# Autodesk Inventor assembly: POM_T5_10
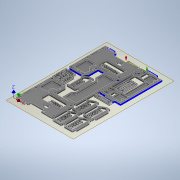
[picture p0: Inventor's stored thumbnail of the model, 180x180]
Saved by Autodesk Inventor 2022 (Build 260153000, 153)
## iProperties
Created: 2022-09-28
Part Number: POM_T5_10
Document SubType Name: Assembly
Designer: Masato
Author: Masato
## Documents named in this file (13)
- C:\Users\ヨコオリク\Documents\CITBrains\SUSTAINA-OP\Cam\POM_T5\POM_T5_10.iam
- C:\Users\ヨコオリク\Documents\CITBrains\SUSTAINA-OP\Cam\DisposableBoard.ipt
- C:\Users\ヨコオリク\Documents\CITBrains\SUSTAINA-OP\UpperBody\Cockpit\Cockpit_back_frame.ipt
- C:\Users\ヨコオリク\Documents\CITBrains\SUSTAINA-OP\UpperBody\Cockpit\Cockpit_battery_back_door.ipt
- C:\Users\ヨコオリク\Documents\CITBrains\SUSTAINA-OP\UpperBody\Cockpit\Cockpit_carrier_board_frame.ipt
- C:\Users\ヨコオリク\Documents\CITBrains\SUSTAINA-OP\UpperBody\Cockpit\Cockpit_side_frame.ipt
- C:\Users\ヨコオリク\Documents\CITBrains\SUSTAINA-OP\UpperBody\Cockpit\Cockpit_side_frame_MIR.ipt
- C:\Users\ヨコオリク\Documents\CITBrains\SUSTAINA-OP\OptionParts\DrillingJigs\Head_neck_diagonal_Jig_back.ipt
- C:\Users\ヨコオリク\Documents\CITBrains\SUSTAINA-OP\OptionParts\DrillingJigs\Head_neck_diagonal_Jig_side.ipt
- C:\Users\ヨコオリク\Documents\CITBrains\SUSTAINA-OP\OptionParts\DrillingJigs\UpperArm_diagonal_Jig.ipt
- C:\Users\ヨコオリク\Documents\CITBrains\SUSTAINA-OP\OptionParts\DrillingJigs\ForeArm_diagonal_Jig_inside.ipt
- C:\Users\ヨコオリク\Documents\CITBrains\SUSTAINA-OP\OptionParts\DrillingJigs\ForeArm_diagonal_Jig_outside.ipt
- C:\Users\ヨコオリク\Documents\CITBrains\SUSTAINA-OP\OptionParts\DrillingJigs\Cockpit_side_frame_Jig.ipt
## Components (24 placed, 12 different names)
1. DisposableBoard:1 — フラッシュ:1, フラッシュ:2, フラッシュ:3, フラッシュ:4, フラッシュ:5, フラッシュ:6, フラッシュ:14, フラッシュ:15, フラッシュ:16
2. Cockpit_back_frame:1 — メイト:5, フラッシュ:12, メイト:18, メイト:19
3. Cockpit_battery_back_door:1 — メイト:3, メイト:12, フラッシュ:10, メイト:13, メイト:15, メイト:24
4. Cockpit_side_frame:1 — メイト:7, フラッシュ:5, フラッシュ:6, フラッシュ:9, メイト:12, フラッシュ:10, 正接:1, メイト:20, 正接:2, メイト:30, メイト:31
5. Cockpit_side_frame_MIR:1 — メイト:11, フラッシュ:9, メイト:13, フラッシュ:12, メイト:33, メイト:34
6. Cockpit_carrier_board_frame:2 — メイト:10, メイト:15, 正接:1, メイト:36, メイト:37
7. Head_neck_diagonal_Jig_side:4 — メイト:21, フラッシュ:15, メイト:22
8. Head_neck_diagonal_Jig_back:3 — メイト:23, メイト:24
9. ForeArm_diagonal_Jig_inside:1 — メイト:29, メイト:30, メイト:31
10. ForeArm_diagonal_Jig_outside:1 — メイト:32, メイト:33, メイト:34
11. Cockpit_side_frame_Jig:1 — メイト:35, メイト:36, メイト:37
12. Head_neck_diagonal_Jig_back:1 — メイト:16, メイト:18, メイト:19
13. Head_neck_diagonal_Jig_back:2
14. Head_neck_diagonal_Jig_side:1 — メイト:17, メイト:20, フラッシュ:14, メイト:22
15. Head_neck_diagonal_Jig_side:2
16. Head_neck_diagonal_Jig_side:3
17. Cockpit_carrier_board_frame:3 — メイト:25, フラッシュ:16, 正接:2, メイト:27, メイト:28
18. Cockpit_carrier_board_frame:4
19. Cockpit_carrier_board_frame:5
20. Cockpit_carrier_board_frame:6
21. UpperArm_diagonal_Jig:1 — メイト:26, メイト:27, メイト:28
22. UpperArm_diagonal_Jig:2
23. UpperArm_diagonal_Jig:3
24. UpperArm_diagonal_Jig:4
## Component patterns: (2 elements, first: Head_neck_diagonal_Jig_back:1), (3 elements, first: Head_neck_diagonal_Jig_side:1), (4 elements, first: Cockpit_carrier_board_frame:3), (4 elements, first: UpperArm_diagonal_Jig:1)
## Relationships (44: Mate 30, Flush 12, Tangent 2)
- フラッシュ:1 [Flush]: DisposableBoard:1
- フラッシュ:2 [Flush]: DisposableBoard:1
- フラッシュ:3 [Flush]: DisposableBoard:1
- フラッシュ:4 [Flush]: DisposableBoard:1
- メイト:3 [Mate]: Cockpit_battery_back_door:1
- メイト:5 [Mate]: Cockpit_back_frame:1
- メイト:7 [Mate]: Cockpit_side_frame:1
- メイト:10 [Mate]: Cockpit_carrier_board_frame:2
- メイト:11 [Mate]: Cockpit_side_frame_MIR:1
- フラッシュ:5 [Flush] (-2 mm): DisposableBoard:1 ↔ Cockpit_side_frame:1
- フラッシュ:6 [Flush] (2 mm): DisposableBoard:1 ↔ Cockpit_side_frame:1
- フラッシュ:9 [Flush]: Cockpit_side_frame:1 ↔ Cockpit_side_frame_MIR:1
- メイト:12 [Mate] (2.1 mm): Cockpit_battery_back_door:1 ↔ Cockpit_side_frame:1
- フラッシュ:10 [Flush]: Cockpit_battery_back_door:1 ↔ Cockpit_side_frame:1
- メイト:13 [Mate] (2.1 mm): Cockpit_battery_back_door:1 ↔ Cockpit_side_frame_MIR:1
- フラッシュ:12 [Flush]: Cockpit_back_frame:1 ↔ Cockpit_side_frame_MIR:1
- メイト:15 [Mate] (2.1 mm): Cockpit_battery_back_door:1 ↔ Cockpit_carrier_board_frame:2
- 正接:1 [Tangent] (2.1 mm): Cockpit_side_frame:1 ↔ Cockpit_carrier_board_frame:2
- メイト:16 [Mate]: Head_neck_diagonal_Jig_back:1
- メイト:17 [Mate]: Head_neck_diagonal_Jig_side:1
- メイト:18 [Mate] (2.1 mm): Cockpit_back_frame:1 ↔ Head_neck_diagonal_Jig_back:1
- メイト:19 [Mate] (2.1 mm): Cockpit_back_frame:1 ↔ Head_neck_diagonal_Jig_back:1
- メイト:20 [Mate] (2.1 mm): Cockpit_side_frame:1 ↔ Head_neck_diagonal_Jig_side:1
- フラッシュ:14 [Flush] (2 mm): DisposableBoard:1 ↔ Head_neck_diagonal_Jig_side:1
- メイト:21 [Mate]: Head_neck_diagonal_Jig_side:4
- フラッシュ:15 [Flush] (2 mm): DisposableBoard:1 ↔ Head_neck_diagonal_Jig_side:4
- メイト:22 [Mate] (2.1 mm): Head_neck_diagonal_Jig_side:4 ↔ Head_neck_diagonal_Jig_side:1
- メイト:23 [Mate]: Head_neck_diagonal_Jig_back:3
- メイト:24 [Mate] (2.1 mm): Cockpit_battery_back_door:1 ↔ Head_neck_diagonal_Jig_back:3
- メイト:25 [Mate]: Cockpit_carrier_board_frame:3
- フラッシュ:16 [Flush] (2 mm): DisposableBoard:1 ↔ Cockpit_carrier_board_frame:3
- 正接:2 [Tangent] (2.1 mm): Cockpit_side_frame:1 ↔ Cockpit_carrier_board_frame:3
- メイト:26 [Mate]: UpperArm_diagonal_Jig:1
- メイト:27 [Mate] (2.1 mm): Cockpit_carrier_board_frame:3 ↔ UpperArm_diagonal_Jig:1
- メイト:28 [Mate] (2.1 mm): Cockpit_carrier_board_frame:3 ↔ UpperArm_diagonal_Jig:1
- メイト:29 [Mate]: ForeArm_diagonal_Jig_inside:1
- メイト:30 [Mate] (2.1 mm): Cockpit_side_frame:1 ↔ ForeArm_diagonal_Jig_inside:1
- メイト:31 [Mate] (2.1 mm): Cockpit_side_frame:1 ↔ ForeArm_diagonal_Jig_inside:1
- メイト:32 [Mate]: ForeArm_diagonal_Jig_outside:1
- メイト:33 [Mate] (2.1 mm): Cockpit_side_frame_MIR:1 ↔ ForeArm_diagonal_Jig_outside:1
- メイト:34 [Mate] (2.1 mm): Cockpit_side_frame_MIR:1 ↔ ForeArm_diagonal_Jig_outside:1
- メイト:35 [Mate]: Cockpit_side_frame_Jig:1
- メイト:36 [Mate] (2.1 mm): Cockpit_carrier_board_frame:2 ↔ Cockpit_side_frame_Jig:1
- メイト:37 [Mate] (2.1 mm): Cockpit_carrier_board_frame:2 ↔ Cockpit_side_frame_Jig:1
